# Autodesk Inventor assembly: Upper
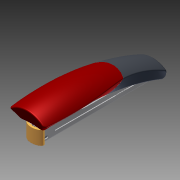
[picture p0: Inventor's stored thumbnail of the model, 180x180]
Saved by Autodesk Inventor 2011 (Build 150239000, 239)
## iProperties
Shininess: 64.0
Length Units: 11272
Angle Units: 11279
Time Units: 11290
Mass Units: 11286
Length Display Precision: 3
Angle Display Precision: 2
Compacted: True
Part Number: Upper
Document SubType Name: Assembly
Created: 2002-09-25
Designer: Autodesk, Inc.
Project: Inventor Samples
Mass: 573.111 g
Surface Area: 569.005 cm^2
Volume: 73.2123 cm^3
Density: 7.82807 g/cm^3
Density: 0.0
Volumn: 0.0
Area: 0.0
PropertySet Name: Model Information
Control State: 0
Master: False
Checked Out: False
Author: Autodesk, Inc.
Revision Number: A
## Documents named in this file (5)
- C:\Users\Public\Documents\Autodesk\Inventor 2011\Samples\Models\Assemblies\Stapler\Components\Upper.iam
- C:\Users\Public\Documents\Autodesk\Inventor 2011\Samples\Models\Assemblies\Stapler\Components\Upper - Back.ipt
- C:\Users\Public\Documents\Autodesk\Inventor 2011\Samples\Models\Assemblies\Stapler\Components\Upper - Front.ipt
- C:\Users\Public\Documents\Autodesk\Inventor 2011\Samples\Models\Assemblies\Stapler\Components\Channel - Spring Clip.ipt
- C:\Users\Public\Documents\Autodesk\Inventor 2011\Samples\Models\Assemblies\Stapler\Components\Channel.iam
## Components (4 placed, 4 different names)
1. Upper - Back:1 — Mate:1, Flush:1, Mate:2, Mate:3, Flush:2, Flush:3, Angle:1, Mate:4
2. Upper - Front:1 — Mate:1, Flush:1, Mate:2
3. Channel - Spring Clip:1 — Mate:3, Flush:2, Mate:5
4. Channel:1 [sub-assembly] — Flush:3, Angle:1, Mate:4, Mate:5
## Relationships (9: Mate 5, Flush 3, Angle 1)
- Mate:1: Upper - Back:1 ↔ Upper - Front:1
- Flush:1: Upper - Back:1 ↔ Upper - Front:1
- Mate:2: Upper - Back:1 ↔ Upper - Front:1
- Mate:3: Upper - Back:1 ↔ Channel - Spring Clip:1
- Flush:2: Upper - Back:1 ↔ Channel - Spring Clip:1
- Flush:3: Upper - Back:1 ↔ Channel:1
- Angle:1 (0 deg): Upper - Back:1 ↔ Channel:1
- Mate:4: Upper - Back:1 ↔ Channel:1
- Mate:5: Channel - Spring Clip:1 ↔ Channel:1
